# Autodesk Inventor assembly: Deltabot - Small Model
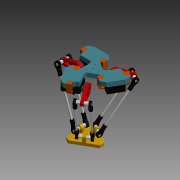
[picture p0: Inventor's stored thumbnail of the model, 180x180]
Saved by Autodesk Inventor 2014 SP1 (Build 180222100, 222)
## iProperties
Created: 2013-12-25
Part Number: Deltabot - Small Model
Document SubType Name: Assembly
Designer: tom
Title: D:\My Documents\Work\GitHub\Delta_Robots\Delatabot - Small Model\Deltabot - Small Model.stp
Creation Date: 2013-12-24
Sending System: ACIS
Author: tom
## Documents named in this file (8)
- C:\Users\tom\Documents\GitHub\Delta_Robots\Delatabot - Small Model\Inventor\Deltabot - Small Model\Deltabot - Small Model.iam
- C:\Users\tom\Documents\GitHub\Delta_Robots\Delatabot - Small Model\Inventor\Deltabot - Small Model\Component8 Copy2.ipt
- C:\Users\tom\Documents\GitHub\Delta_Robots\Delatabot - Small Model\Inventor\Deltabot - Small Model\Servo Mechanism.iam
- C:\Users\tom\Documents\GitHub\Delta_Robots\Delatabot - Small Model\Inventor\Deltabot - Small Model\Upper Arm.iam
- C:\Users\tom\Documents\GitHub\Delta_Robots\Delatabot - Small Model\Inventor\Deltabot - Small Model\Arm Rod.iam
- C:\Users\tom\Documents\GitHub\Delta_Robots\Delatabot - Small Model\Inventor\Deltabot - Small Model\Screw 6-32.ipt
- C:\Users\tom\Documents\GitHub\Delta_Robots\Delatabot - Small Model\Inventor\Deltabot - Small Model\Bearing.ipt
- C:\Users\tom\Documents\GitHub\Delta_Robots\Delatabot - Small Model\Inventor\Deltabot - Small Model\Lower Platform.iam
## Components (27 placed, 7 different names)
1. Upper Platform — Mate:1, Mate:2, Mate:3, Mate:4, Mate:5, Mate:6, Mate:7, Mate:8, Mate:9
2. Servo Mechanism:1 [sub-assembly] — Mate:1, Mate:2, Mate:3, Rotational:1
3. Upper Arm:1 [sub-assembly] — Rotational:1, Rotational:8, Rotational:10
4. Servo Mechanism:2 [sub-assembly] — Mate:4, Mate:5, Mate:6, Rotational:2
5. Upper Arm:2 [sub-assembly] — Rotational:2, Rotational:13, Rotational:14
6. Servo Mechanism:3 [sub-assembly] — Mate:7, Mate:8, Mate:9, Rotational:3
7. Upper Arm:3 [sub-assembly] — Rotational:3, Mate:10, Mate:11, Rotational:4, Rotational:6
8. Arm Rod:2 [sub-assembly] — Ball:1, Ball:2
9. Screw 6-32:1 — Mate:10, Mate:11
10. Bearing:1 — Rotational:4, Ball:1
11. Lower Platform:2 [sub-assembly] — Rotational:5, Rotational:7, Rotational:9, Rotational:11, Rotational:12, Rotational:15
12. Bearing:2 — Ball:2, Rotational:5
13. Bearing:3 — Ball:4, Rotational:6
14. Bearing:4 — Ball:3, Rotational:7
15. Arm Rod:3 [sub-assembly] — Ball:3, Ball:4
16. Bearing:5 — Rotational:8, Ball:5
17. Bearing:6 — Rotational:9, Ball:6
18. Arm Rod:4 [sub-assembly] — Ball:5, Ball:6
19. Bearing:7 — Rotational:10, Ball:7
20. Bearing:8 — Rotational:11, Ball:8
21. Arm Rod:5 [sub-assembly] — Ball:7, Ball:8
22. Bearing:9 — Rotational:15, Ball:10
23. Bearing:10 — Rotational:14, Ball:9
24. Bearing:11 — Rotational:13, Ball:11
25. Bearing:12 — Rotational:12, Ball:12
26. Arm Rod:6 [sub-assembly] — Ball:9, Ball:10
27. Arm Rod:7 [sub-assembly] — Ball:11, Ball:12
## Relationships (38: RevoluteJoint 15, BallJoint 12, Mate 11)
- Mate:1: Upper Platform ↔ Servo Mechanism:1
- Mate:2: Upper Platform ↔ Servo Mechanism:1
- Mate:3: Upper Platform ↔ Servo Mechanism:1
- Mate:4: Upper Platform ↔ Servo Mechanism:2
- Mate:5: Upper Platform ↔ Servo Mechanism:2
- Mate:6: Upper Platform ↔ Servo Mechanism:2
- Mate:7: Upper Platform ↔ Servo Mechanism:3
- Mate:8: Upper Platform ↔ Servo Mechanism:3
- Mate:9: Upper Platform ↔ Servo Mechanism:3
- Rotational:1 [RevoluteJoint]: Servo Mechanism:1 ↔ Upper Arm:1
- Rotational:2 [RevoluteJoint]: Servo Mechanism:2 ↔ Upper Arm:2
- Rotational:3 [RevoluteJoint]: Servo Mechanism:3 ↔ Upper Arm:3
- Mate:10: Upper Arm:3 ↔ Screw 6-32:1
- Mate:11 (5.5 mm): Upper Arm:3 ↔ Screw 6-32:1
- Rotational:4 [RevoluteJoint]: Upper Arm:3 ↔ Bearing:1
- Ball:1: Arm Rod:2 ↔ Bearing:1
- Ball:2: Arm Rod:2 ↔ Bearing:2
- Rotational:5 [RevoluteJoint]: Lower Platform:2 ↔ Bearing:2
- Ball:3: Bearing:4 ↔ Arm Rod:3
- Ball:4: Bearing:3 ↔ Arm Rod:3
- Rotational:6 [RevoluteJoint]: Upper Arm:3 ↔ Bearing:3
- Rotational:7 [RevoluteJoint]: Lower Platform:2 ↔ Bearing:4
- Rotational:8 [RevoluteJoint]: Upper Arm:1 ↔ Bearing:5
- Rotational:9 [RevoluteJoint]: Lower Platform:2 ↔ Bearing:6
- Ball:5: Bearing:5 ↔ Arm Rod:4
- Ball:6: Bearing:6 ↔ Arm Rod:4
- Rotational:10 [RevoluteJoint]: Upper Arm:1 ↔ Bearing:7
- Rotational:11 [RevoluteJoint]: Lower Platform:2 ↔ Bearing:8
- Ball:7: Bearing:7 ↔ Arm Rod:5
- Ball:8: Bearing:8 ↔ Arm Rod:5
- Rotational:12 [RevoluteJoint]: Lower Platform:2 ↔ Bearing:12
- Rotational:13 [RevoluteJoint]: Upper Arm:2 ↔ Bearing:11
- Rotational:14 [RevoluteJoint]: Upper Arm:2 ↔ Bearing:10
- Rotational:15 [RevoluteJoint]: Lower Platform:2 ↔ Bearing:9
- Ball:9: Bearing:10 ↔ Arm Rod:6
- Ball:10: Bearing:9 ↔ Arm Rod:6
- Ball:11: Bearing:11 ↔ Arm Rod:7
- Ball:12: Bearing:12 ↔ Arm Rod:7
